# Autodesk Inventor assembly: Prototype
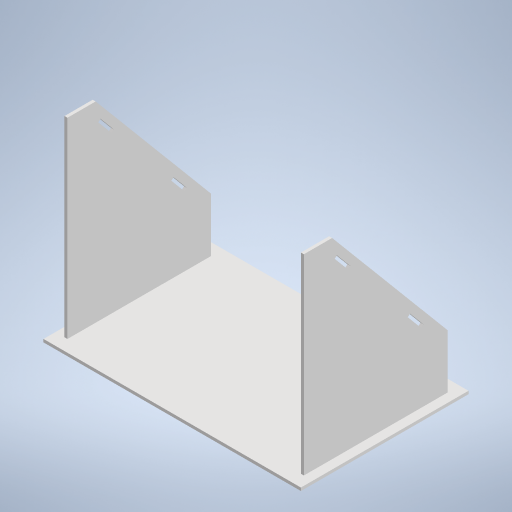
[picture p0: Inventor's stored thumbnail of the model, 512x512]
Saved by Autodesk Inventor 2024 (Build 280153000, 153)
## iProperties
Created: 2023-11-07
Part Number: Prototype
Document SubType Name: Assembly
Designer: flynf
Author: flynf
## Documents named in this file (3)
- C:\Users\flynf\Documents\Prototype.iam
- C:\Users\flynf\Documents\C4Base.ipt
- C:\Users\flynf\Documents\C4Side.ipt
## Components (3 placed, 2 different names)
1. C4Base:1 — Mate:1, Flush:1, Mate:2, Mate:3, Flush:2, Flush:3
2. C4Side:1 — Mate:1, Flush:1, Mate:2
3. C4Side:2 — Mate:3, Flush:2, Flush:3
## Relationships (6: Mate 3, Flush 3)
- Mate:1: C4Base:1 ↔ C4Side:1
- Flush:1: C4Base:1 ↔ C4Side:1
- Mate:2: C4Base:1 ↔ C4Side:1
- Mate:3: C4Base:1 ↔ C4Side:2
- Flush:2: C4Base:1 ↔ C4Side:2
- Flush:3 (12.7 mm): C4Base:1 ↔ C4Side:2
